# Autodesk Inventor assembly: Sestava1
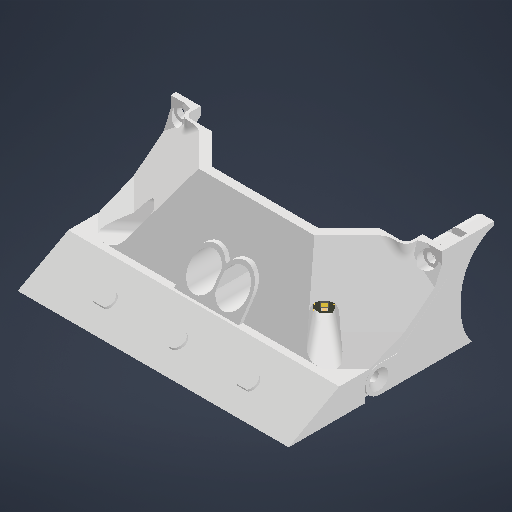
[picture p0: Inventor's stored thumbnail of the model, 512x512]
Saved by Autodesk Inventor 2025 (Build 290162000, 162)
## iProperties
Created: 2024-10-19
Part Number: Sestava1
Document SubType Name: Assembly
Designer: Simak
Author: Simak
## Documents named in this file (5)
- C:\_desktop\GitHub\Sumec-MiniSumo\-3D-\Sestava1.iam
- C:\_desktop\GitHub\Sumec-MiniSumo\-3D-\3D_printed\body-main.ipt
- C:\_desktop\GitHub\Sumec-MiniSumo\-3D-\3D_printed\body-front.ipt
- C:\_desktop\GitHub\Sumec-MiniSumo\-3D-\electronics\pololu-digital-distance-sensor-irs17a.ipt
- C:\_desktop\GitHub\Sumec-MiniSumo\-3D-\electronics\AssemBeneWake TF-LUNA.ipt
## Components (4 placed, 4 different names)
1. body-main:1 — OPEN, Stejný směr:1, Vložit:1
2. body-front:1 — OPEN, Stejný směr:1, Vložit:1, Stejný směr:2, Proti sobě:2, Proti sobě:3, Proti sobě:4
3. pololu-digital-distance-sensor-irs17a:1 — Stejný směr:2, Proti sobě:2, Proti sobě:3
4. AssemBeneWake TF-LUNA:1 — Proti sobě:4
## Relationships (7: Mate 4, Flush 2, Insert 1)
- OPEN [Mate]: body-main:1 ↔ body-front:1
- Stejný směr:1 [Flush]: body-main:1 ↔ body-front:1
- Vložit:1 [Insert]: body-main:1 ↔ body-front:1
- Stejný směr:2 [Flush]: body-front:1 ↔ pololu-digital-distance-sensor-irs17a:1
- Proti sobě:2 [Mate]: body-front:1 ↔ pololu-digital-distance-sensor-irs17a:1
- Proti sobě:3 [Mate]: body-front:1 ↔ pololu-digital-distance-sensor-irs17a:1
- Proti sobě:4 [Mate]: body-front:1 ↔ AssemBeneWake TF-LUNA:1
